# Autodesk Inventor assembly: Assembly5 (Valve Sub Assembly)
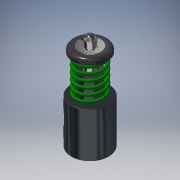
[picture p0: Inventor's stored thumbnail of the model, 180x180]
Saved by Autodesk Inventor 2018 (Build 220112000, 112)
## iProperties
Created: 2023-04-19
Part Number: Assembly5 (Valve Sub Assembly)
Document SubType Name: Assembly
Designer: Habib Mohamed
Author: Habib Mohamed
## Documents named in this file (6)
- D:\Inventor\My projects\Rotary Engine\Assembly\Assembly5 (Valve Sub Assembly).iam
- D:\Inventor\My projects\Rotary Engine\Component 15 (Hold Down Valve Spring).ipt
- D:\Inventor\My projects\Rotary Engine\Component 23 (Valve Spring).ipt
- D:\Inventor\My projects\Rotary Engine\Component 24 (Valve).ipt
- D:\Inventor\My projects\Rotary Engine\Component 26 (Valve Cup).ipt
- C:\Users\Habib Mohamed\Documents\Inventor\Content Center Files\R2018\en-US\DIN 6799\DIN 6799 - 2.3 3.ipt
## Components (5 placed, 5 different names)
1. Component 15 (Hold Down Valve Spring):1 — Mate:3, Flush:1, Mate:5
2. Component 23 (Valve Spring):1 — Mate:4, Mate:5
3. Component 24 (Valve):1 — Mate:2, Mate:3, Flush:1, Mate:4, Valve offset, Mate:6, Mate:7
4. Component 26 (Valve Cup):1 — Mate:1, Mate:2, Valve offset
5. DIN 6799 2.3:1 — Mate:6, Mate:7
## Relationships (9: Mate 7, Flush 2)
- Mate:1: Component 26 (Valve Cup):1
- Mate:2: Component 24 (Valve):1 ↔ Component 26 (Valve Cup):1
- Mate:3: Component 15 (Hold Down Valve Spring):1 ↔ Component 24 (Valve):1
- Flush:1: Component 15 (Hold Down Valve Spring):1 ↔ Component 24 (Valve):1
- Mate:4: Component 23 (Valve Spring):1 ↔ Component 24 (Valve):1
- Valve offset [Flush]: Component 24 (Valve):1 ↔ Component 26 (Valve Cup):1
- Mate:5: Component 15 (Hold Down Valve Spring):1 ↔ Component 23 (Valve Spring):1
- Mate:6: Component 24 (Valve):1 ↔ DIN 6799 2.3:1
- Mate:7: Component 24 (Valve):1 ↔ DIN 6799 2.3:1
